# Autodesk Inventor assembly: 000000
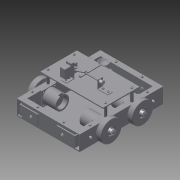
[picture p0: Inventor's stored thumbnail of the model, 180x180]
Saved by Autodesk Inventor 2015 (Build 190159000, 159)
## iProperties
Created: 2015-05-30
Part Number: 000000
Document SubType Name: Assembly
Designer: Wesley
Author: Wesley
## Documents named in this file (4)
- C:\Users\Wesley\Documents\GitHub\EngineeringFinal\Engineering\Engineering Documentation\CADS\00__00\000000.iam
- C:\Users\Wesley\Documents\GitHub\EngineeringFinal\Engineering\Engineering Documentation\CADS\0001__\000100.iam
- C:\Users\Wesley\Documents\GitHub\EngineeringFinal\Engineering\Engineering Documentation\CADS\0002__\000200.iam
- C:\Users\Wesley\Documents\GitHub\EngineeringFinal\Engineering\Engineering Documentation\CADS\0001__\000105-2.ipt
## Components (6 placed, 3 different names)
1. 000100:1 [sub-assembly] — Mate:1, Mate:2, Mate:3, Mate:4, Mate:5, Mate:6, Mate:7, Mate:8, Mate:9, Mate:10, Mate:11
2. 000200:1 [sub-assembly] — Mate:1, Mate:2, Mate:3
3. 000105-2:1 — Mate:6, Mate:7
4. 000105-2:2 — Mate:4, Mate:5
5. 000105-2:3 — Mate:8, Mate:11
6. 000105-2:4 — Mate:9, Mate:10
## Relationships (11: Mate 11)
- Mate:1: 000100:1 ↔ 000200:1
- Mate:2: 000100:1 ↔ 000200:1
- Mate:3: 000100:1 ↔ 000200:1
- Mate:4: 000100:1 ↔ 000105-2:2
- Mate:5: 000100:1 ↔ 000105-2:2
- Mate:6: 000100:1 ↔ 000105-2:1
- Mate:7: 000100:1 ↔ 000105-2:1
- Mate:8: 000100:1 ↔ 000105-2:3
- Mate:9: 000100:1 ↔ 000105-2:4
- Mate:10: 000100:1 ↔ 000105-2:4
- Mate:11: 000100:1 ↔ 000105-2:3
